# Autodesk Inventor assembly: 2XL-430montado
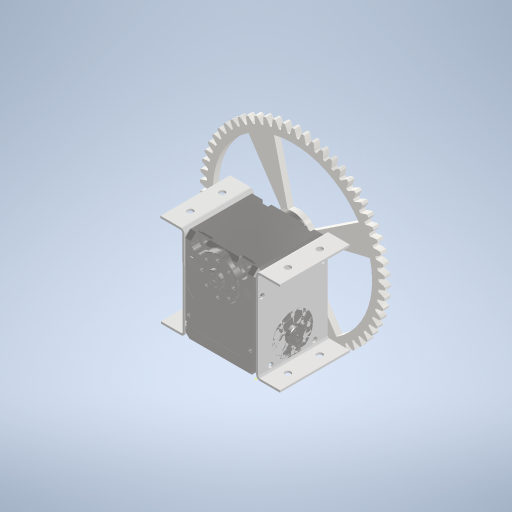
[picture p0: Inventor's stored thumbnail of the model, 512x512]
Saved by Autodesk Inventor 2023 (Build 270158000, 158)
## iProperties
Created: 2019-05-16
Part Number: 2XL-430montado
Document SubType Name: Assembly
Designer: hiago.sodre
Sending System: CREO PARAMETRIC BY PTC INC, 2018260
Preprocessor: CREO PARAMETRIC BY PTC INC, 2018260
Title: DC14_A01_REF_ASM
Author: eum
Revision Number: 5LAST_VERSION
## Documents named in this file (11)
- C:\Users\hiago.sodre\Downloads\ssl_CAD-main\SSLurubots\2XL-430montado.iam
- C:\Users\hiago.sodre\Downloads\ssl_CAD-main\SSLurubots\DC14_A01_REF.ipt
- C:\Users\hiago.sodre\Downloads\ssl_CAD-main\SSLurubots\S3B-EH.ipt
- C:\Users\hiago.sodre\Downloads\ssl_CAD-main\SSLurubots\EHR-3.ipt
- C:\Users\hiago.sodre\Downloads\ssl_CAD-main\SSLurubots\PHS_M2X33_TAP_K.ipt
- C:\Users\hiago.sodre\Downloads\ssl_CAD-main\SSLurubots\DC14_A01_INSERT_2.ipt
- C:\Users\hiago.sodre\Downloads\ssl_CAD-main\SSLurubots\DC14_A01_INSERT_1.ipt
- C:\Users\hiago.sodre\Downloads\ssl_CAD-main\SSLurubots\DC11_A01_HORN_REF_ASM.iam
- C:\Users\hiago.sodre\Downloads\ssl_CAD-main\SSLurubots\DC11_A01_IDLER_REF_ASM.iam
- C:\Users\hiago.sodre\Downloads\ssl_CAD-main\SSLurubots\Suportmotor.ipt
- C:\Users\hiago.sodre\Downloads\ssl_CAD-main\SSLurubots\Engrenaje.iam
## Components (26 placed, 25 different names)
1. 68 — Rígida:1, Rígida:2, Rotativa:2
2. 69
3. 70
4. 71
5. 72
6. 73
7. 74
8. 75
9. 76
10. 77
11. 78
12. 79
13. 80
14. 81
15. 82
16. 83
17. 84
18. 85
19. 86
20. 89 [sub-assembly]
21. 90 [sub-assembly]
22. 94 [sub-assembly]
23. 95 [sub-assembly] — Rotativa:1, Rotativa:2
24. Suportmotor:1 — Rígida:1
25. Suportmotor:2 — Rígida:2
26. Engrenaje:1 [sub-assembly] — Rotativa:1
## Relationships (4: WeldJoint 2, RevoluteJoint 2)
- Rígida:1 [WeldJoint]: 68 ↔ Suportmotor:1
- Rígida:2 [WeldJoint]: 68 ↔ Suportmotor:2
- Rotativa:1 [RevoluteJoint]: 95 ↔ Engrenaje:1
- Rotativa:2 [RevoluteJoint]: 68 ↔ 95
